# Autodesk Inventor assembly: Ensamble_1
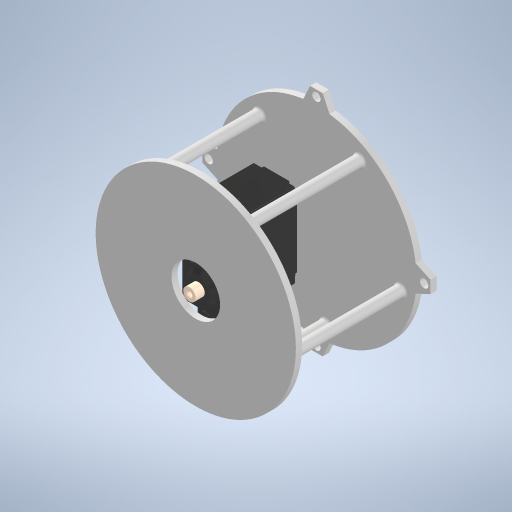
[picture p0: Inventor's stored thumbnail of the model, 512x512]
Saved by Autodesk Inventor 2023 (Build 270158000, 158)
## iProperties
Created: 2024-09-27
Part Number: Ensamble_1
Document SubType Name: Assembly
Designer: sebas
Author: sebas
## Documents named in this file (3)
- C:\Users\sebas\OneDrive\Documentos\ILLERO_MODELADO_ROBOT\Ensamble_1.iam
- C:\Users\sebas\OneDrive\Documentos\ILLERO_MODELADO_ROBOT\Pieza_base_1.ipt
- C:\Users\sebas\OneDrive\Documentos\ILLERO_MODELADO_ROBOT\User Library-Subasa Servo S3003.ipt
## Components (2 placed, 2 different names)
1. Pieza_base_1:1 — Coincidencia:17, Coincidencia:18, Coincidencia:19
2. User Library-Subasa Servo S3003:4 — Coincidencia:17, Coincidencia:19
## Relationships (3: Mate 3)
- Coincidencia:17 [Mate]: Pieza_base_1:1 ↔ User Library-Subasa Servo S3003:4
- Coincidencia:18 [Mate]: Pieza_base_1:1
- Coincidencia:19 [Mate]: Pieza_base_1:1 ↔ User Library-Subasa Servo S3003:4
